# Autodesk Inventor assembly: Assembly_Cube_Laserblock_v3
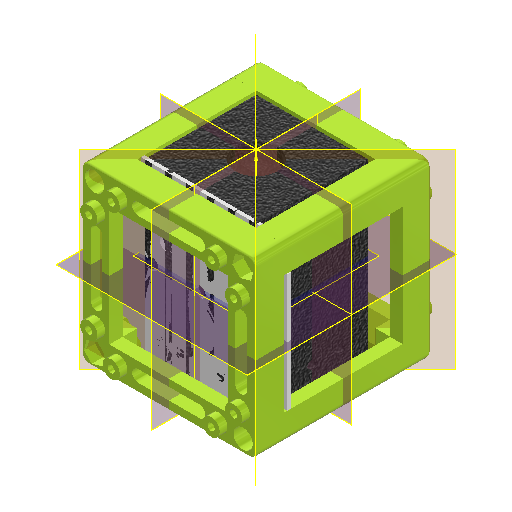
[picture p0: Inventor's stored thumbnail of the model, 512x512]
Saved by Autodesk Inventor 2023 (Build 270158000, 158)
## iProperties
Created: 2023-04-07
Part Number: Assembly_Cube_Laserblock_v3
Document SubType Name: Assembly
Designer: diederichbenedict
Author: diederichbenedict
## Documents named in this file (4)
- C:\Users\diederichbenedict\Downloads\UC2 setup design\UC2 setup design\Assembly_Cube_Laserblock_v3.iam
- C:\Users\diederichbenedict\Downloads\UC2 setup design\UC2 setup design\Assembly_Cube_empty_IM_v3.iam
- C:\Users\diederichbenedict\Downloads\UC2 setup design\UC2 setup design\00_LASER_640nm.ipt
- C:\Users\diederichbenedict\Downloads\UC2 setup design\UC2 setup design\20_Cube_insert_Laser_Block_adjustable_v3.ipt
## Components (3 placed, 3 different names)
1. Assembly_Cube_empty_IM_v3:1 [sub-assembly] — Mate:1, Angle:1, Mate:2, Flush:2, Flush:3
2. 20_Cube_insert_Laser_Block_adjustable_v3:1 — Flush:1, Flush:2, Flush:3
3. 00_LASER_640nm:1 — Mate:1, Angle:1, Mate:2, Flush:1
## Relationships (6: Flush 3, Mate 2, Angle 1)
- Mate:1: Assembly_Cube_empty_IM_v3:1 ↔ 00_LASER_640nm:1
- Angle:1 (0 deg): Assembly_Cube_empty_IM_v3:1 ↔ 00_LASER_640nm:1
- Mate:2: Assembly_Cube_empty_IM_v3:1 ↔ 00_LASER_640nm:1
- Flush:1: 20_Cube_insert_Laser_Block_adjustable_v3:1 ↔ 00_LASER_640nm:1
- Flush:2: Assembly_Cube_empty_IM_v3:1 ↔ 20_Cube_insert_Laser_Block_adjustable_v3:1
- Flush:3: Assembly_Cube_empty_IM_v3:1 ↔ 20_Cube_insert_Laser_Block_adjustable_v3:1
